# Autodesk Inventor assembly: RaspberryPi_Encloser
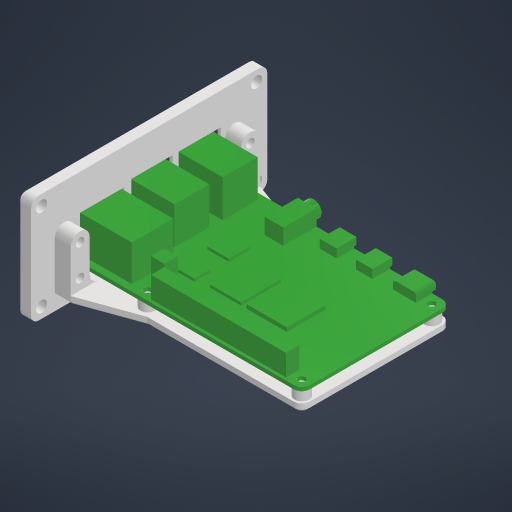
[picture p0: Inventor's stored thumbnail of the model, 512x512]
Saved by Autodesk Inventor 2024 (Build 280153000, 153)
## iProperties
Created: 2025-09-25
Part Number: RaspberryPi_Encloser
Document SubType Name: Assembly
Designer: kevin
Author: kevin
## Documents named in this file (4)
- C:\Users\kevin\Desktop\SeniorDesign\Head_V3\RaspberryPi_Encloser.iam
- C:\Users\kevin\Desktop\SeniorDesign\RaspberryPi4.ipt
- C:\Users\kevin\Desktop\SeniorDesign\Head_V3\RaspberryPi_baseplate.ipt
- C:\Users\kevin\Desktop\SeniorDesign\Head_V3\RaspberryPi_IO_Shield.ipt
## Components (3 placed, 3 different names)
1. RaspberryPi4:1 — Flush:1
2. RaspberryPi_baseplate:1 — Flush:1, Flush:2, Flush:3
3. RaspberryPi_IO_Shield:1 — Flush:2, Flush:3
## Relationships (3: Flush 3)
- Flush:1: RaspberryPi4:1 ↔ RaspberryPi_baseplate:1
- Flush:2: RaspberryPi_baseplate:1 ↔ RaspberryPi_IO_Shield:1
- Flush:3: RaspberryPi_baseplate:1 ↔ RaspberryPi_IO_Shield:1
